# Autodesk Inventor assembly: V4 Assembly
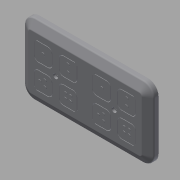
[picture p0: Inventor's stored thumbnail of the model, 180x180]
Saved by Autodesk Inventor 2020 (Build 240168000, 168)
## iProperties
Created: 2020-01-10
Part Number: V4 Assembly
Document SubType Name: Assembly
Designer: user
Author: user
## Documents named in this file (4)
- D:\Documents\Github\Arduino-MiLightHub_switch\3D\V4.2 Assembly.iam
- D:\Documents\Github\Arduino-MiLightHub_switch\3D\V4.2 Plate dual.ipt
- D:\Documents\Github\Arduino-MiLightHub_switch\3D\V4.2 In wall.ipt
- D:\Documents\Github\Arduino-MiLightHub_switch\3D\V4.2 Plate single.ipt
## Components (3 placed, 3 different names)
1. V4.2 In wall:1 — Angle:1, Mate:4, Mate:5, Flush:5, Mate:6, Mate:7, Flush:6
2. V4.2 Plate dual:1 — Flush:2, Flush:3, Mate:5, Flush:6
3. V4.2 Plate single:1 — Flush:2, Flush:3, Angle:1, Mate:4
## Relationships (9: Flush 4, Mate 4, Angle 1)
- Flush:2: V4.2 Plate dual:1 ↔ V4.2 Plate single:1
- Flush:3: V4.2 Plate dual:1 ↔ V4.2 Plate single:1
- Angle:1 (0 deg): V4.2 In wall:1 ↔ V4.2 Plate single:1
- Mate:4: V4.2 In wall:1 ↔ V4.2 Plate single:1
- Mate:5: V4.2 In wall:1 ↔ V4.2 Plate dual:1
- Flush:5: V4.2 In wall:1
- Mate:6: V4.2 In wall:1
- Mate:7: V4.2 In wall:1
- Flush:6: V4.2 In wall:1 ↔ V4.2 Plate dual:1
